# Autodesk Inventor assembly: rodAndKey
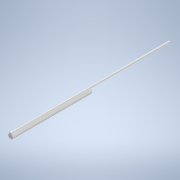
[picture p0: Inventor's stored thumbnail of the model, 180x180]
Saved by Autodesk Inventor 2020.2 (Build 242310000, 310)
## iProperties
Created: 2019-12-09
Part Number: rodAndKey
Document SubType Name: Assembly
Designer: robst
Author: robst
## Documents named in this file (3)
- C:\git\CAD-Development\robSteele\liftSpool\rodAndKey.iam
- C:\git\CAD-Development\robSteele\liftSpool\1497K500_FULLY KEYED 1045 STEEL DRIVE SHAFT.ipt
- C:\git\CAD-Development\robSteele\liftSpool\98491A098_OVERSIZED STEEL MACHINE KEY STOCK.ipt
## Components (2 placed, 2 different names)
1. 1497K500_FULLY KEYED 1045 STEEL DRIVE SHAFT:1 — Mate:1, Flush:1
2. 98491A098_OVERSIZED STEEL MACHINE KEY STOCK:1 — Mate:1, Flush:1
## Relationships (2: Mate 1, Flush 1)
- Mate:1: 1497K500_FULLY KEYED 1045 STEEL DRIVE SHAFT:1 ↔ 98491A098_OVERSIZED STEEL MACHINE KEY STOCK:1
- Flush:1: 1497K500_FULLY KEYED 1045 STEEL DRIVE SHAFT:1 ↔ 98491A098_OVERSIZED STEEL MACHINE KEY STOCK:1
